# Autodesk Inventor assembly: Assembly1
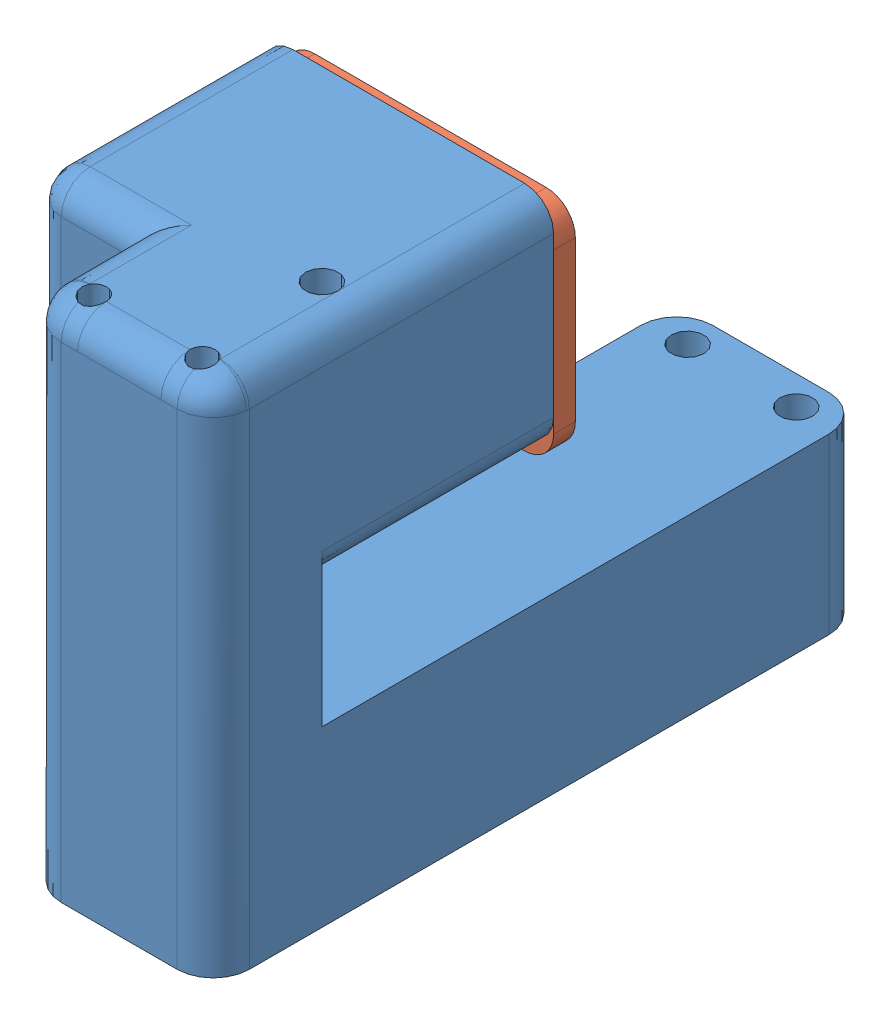
[picture p0: shaded view drawn from the part files that the assembly names]
Saved by Autodesk Inventor 2024.1 (Build 281209000, 209)
## iProperties
Created: 2025-01-19
Part Number: Assembly1
Document SubType Name: Assembly
Designer: Vibhu Iyer
Author: Vibhu Iyer
## Documents named in this file (3)
- C:\Users\thevizwiz\Documents\_Documents Unsynced\projects\motorcycle-alarm\cad\Assembly1.iam
- C:\Users\thevizwiz\Documents\_Documents Unsynced\projects\motorcycle-alarm\cad\button_holder.ipt
- C:\Users\thevizwiz\Documents\_Documents Unsynced\projects\motorcycle-alarm\cad\button_holder_face.ipt
## Components (2 placed, 2 different names)
1. button_holder:1 — Flush:1
2. button_holder_face:1 — Flush:1
## Relationships (1: Flush 1)
- Flush:1: button_holder:1 ↔ button_holder_face:1
